# Autodesk Inventor assembly: Assembly1
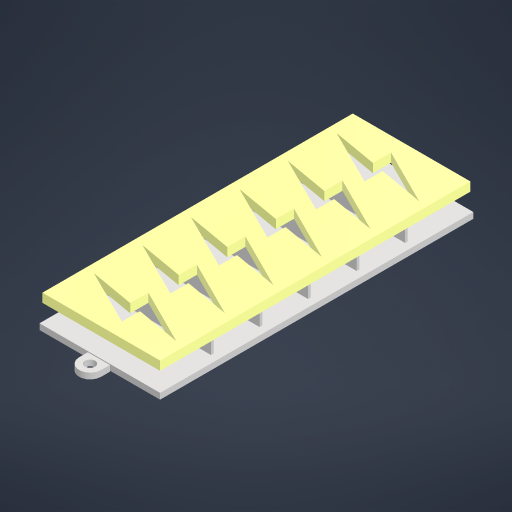
[picture p0: Inventor's stored thumbnail of the model, 512x512]
Saved by Autodesk Inventor 2024.3 (Build 283343000, 343)
## iProperties
Created: 2025-08-06
Part Number: Assembly1
Document SubType Name: Assembly
Designer: giuseppe
Author: giuseppe
## Documents named in this file (4)
- C:\Users\giuseppe\Desktop\Buckshot-Ruolette\CAD\counter\Assembly1.iam
- C:\Users\giuseppe\Desktop\Buckshot-Ruolette\CAD\counter\panel.ipt
- C:\Users\giuseppe\Desktop\Buckshot-Ruolette\CAD\counter\flat base.ipt
- C:\Users\giuseppe\Desktop\Buckshot-Ruolette\CAD\counter\light fixture.ipt
## Components (3 placed, 3 different names)
1. panel:1 — Flush:1, Flush:2
2. flat base:1 — Flush:1, Flush:2, Flush:3, Flush:4
3. light fixture:1 — Flush:3, Flush:4
## Relationships (4: Flush 4)
- Flush:1: panel:1 ↔ flat base:1
- Flush:2: panel:1 ↔ flat base:1
- Flush:3: flat base:1 ↔ light fixture:1
- Flush:4 (6 mm): flat base:1 ↔ light fixture:1
